# Autodesk Inventor assembly: Benchtop-mesoSPIM-Draft
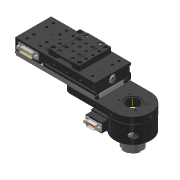
[picture p0: Inventor's stored thumbnail of the model, 180x180]
Saved by Autodesk Inventor 2019 (Build 230136000, 136)
## iProperties
Created: 2020-05-09
Part Number: Benchtop-mesoSPIM-Draft
Document SubType Name: Assembly
Designer: voigt
Author: voigt
## Documents named in this file (5)
- J:\Microscope_Design\CAD_Files\mesoSPIM_design_benchtop_V1\library\ASI\Benchtop-mesoSPIM-Draft.iam
- J:\Microscope_Design\CAD_Files\mesoSPIM_design_benchtop_V1\library\ASI\C60-3060-CMR-1011 - C-MOUNT TO LS50 SLIDE ADAPTER.ipt
- J:\Microscope_Design\CAD_Files\mesoSPIM_design_benchtop_V1\library\ASI\C60-3060-CMR - 3060 C-MOUNT ROTATING ASSEMBLY_C60-3060-CMR-Mo-ER20.iam
- J:\Microscope_Design\CAD_Files\mesoSPIM_design_benchtop_V1\library\ASI\LS-50 LE ASSEMBLY_HOME.iam
- J:\Microscope_Design\CAD_Files\mesoSPIM_design_benchtop_V1\library\ASI\VTS-2112 DOVE RACK ASSEMBLY - (#DV6010 and #DV6020)_DV6010 ASSEMBLY with CDZ-SLIDE C.iam
## Components (4 placed, 4 different names)
1. C60-3060-CMR-1011 - C-MOUNT TO LS50 SLIDE ADAPTER:1 — Mate:3, Flush:1, Mate:4, Mate:5, Mate:6, Angle:1, Mate:7, Mate:8, Mate:9
2. C60-3060-CMR - 3060 C-MOUNT ROTATING ASSEMBLY_C60-3060-CMR-Mo-ER20:1 [sub-assembly] — Mate:4, Mate:5, Mate:6, Angle:1
3. LS-50 LE ASSEMBLY_HOME:1 [sub-assembly] — Mate:7, Mate:8, Mate:9, Mate:10, Mate:11, Mate:12
4. VTS-2112 DOVE RACK ASSEMBLY - (#DV6010 and #DV6020)_DV6010 ASSEMBLY with CDZ-SLIDE C:1 [sub-assembly] — Mate:10, Mate:11, Mate:12
## Relationships (14: Mate 12, Flush 1, Angle 1)
- Mate:1
- Mate:2
- Mate:3: C60-3060-CMR-1011 - C-MOUNT TO LS50 SLIDE ADAPTER:1
- Flush:1: C60-3060-CMR-1011 - C-MOUNT TO LS50 SLIDE ADAPTER:1
- Mate:4: C60-3060-CMR-1011 - C-MOUNT TO LS50 SLIDE ADAPTER:1 ↔ C60-3060-CMR - 3060 C-MOUNT ROTATING ASSEMBLY_C60-3060-CMR-Mo-ER20:1
- Mate:5: C60-3060-CMR-1011 - C-MOUNT TO LS50 SLIDE ADAPTER:1 ↔ C60-3060-CMR - 3060 C-MOUNT ROTATING ASSEMBLY_C60-3060-CMR-Mo-ER20:1
- Mate:6: C60-3060-CMR-1011 - C-MOUNT TO LS50 SLIDE ADAPTER:1 ↔ C60-3060-CMR - 3060 C-MOUNT ROTATING ASSEMBLY_C60-3060-CMR-Mo-ER20:1
- Angle:1 (0 deg): C60-3060-CMR-1011 - C-MOUNT TO LS50 SLIDE ADAPTER:1 ↔ C60-3060-CMR - 3060 C-MOUNT ROTATING ASSEMBLY_C60-3060-CMR-Mo-ER20:1
- Mate:7: C60-3060-CMR-1011 - C-MOUNT TO LS50 SLIDE ADAPTER:1 ↔ LS-50 LE ASSEMBLY_HOME:1
- Mate:8: C60-3060-CMR-1011 - C-MOUNT TO LS50 SLIDE ADAPTER:1 ↔ LS-50 LE ASSEMBLY_HOME:1
- Mate:9: C60-3060-CMR-1011 - C-MOUNT TO LS50 SLIDE ADAPTER:1 ↔ LS-50 LE ASSEMBLY_HOME:1
- Mate:10: LS-50 LE ASSEMBLY_HOME:1 ↔ VTS-2112 DOVE RACK ASSEMBLY - (#DV6010 and #DV6020)_DV6010 ASSEMBLY with CDZ-SLIDE C:1
- Mate:11: LS-50 LE ASSEMBLY_HOME:1 ↔ VTS-2112 DOVE RACK ASSEMBLY - (#DV6010 and #DV6020)_DV6010 ASSEMBLY with CDZ-SLIDE C:1
- Mate:12: LS-50 LE ASSEMBLY_HOME:1 ↔ VTS-2112 DOVE RACK ASSEMBLY - (#DV6010 and #DV6020)_DV6010 ASSEMBLY with CDZ-SLIDE C:1
